# Autodesk Inventor assembly: Servo_DS3218MG_2
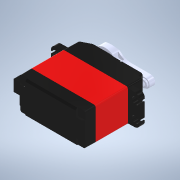
[picture p0: Inventor's stored thumbnail of the model, 180x180]
Saved by Autodesk Inventor 2022 (Build 260153000, 153)
## iProperties
Created: 2020-12-04
Part Number: Servo_DS3218MG_2
Document SubType Name: Assembly
Designer: YusukeKunita
Author: YusukeKunita
## Documents named in this file (3)
- C:\Users\YusukeKunita\Documents\GrabCAD\NHK2022\BasicParts\ServoMotor\Servo_DS3218MG\Servo_DS3218MG_2.iam
- C:\Users\YusukeKunita\Documents\GrabCAD\NHK2022\BasicParts\ServoMotor\Servo_DS3218MG\DS3218MG.ipt
- C:\Users\YusukeKunita\Documents\GrabCAD\NHK2022\BasicParts\ServoMotor\Servo_DS3218MG\Servo_arm_25T.ipt
## Components (2 placed, 2 different names)
1. DS3218MG:1 — 回転:1
2. Servo_arm_25T:1 — 回転:1
## Relationships (1: RevoluteJoint 1)
- 回転:1 [RevoluteJoint] (1.5 mm): DS3218MG:1 ↔ Servo_arm_25T:1
